# Autodesk Inventor assembly: leg_right
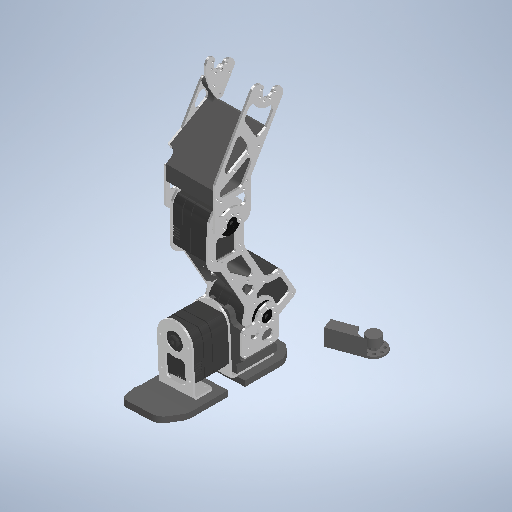
[picture p0: Inventor's stored thumbnail of the model, 512x512]
Saved by Autodesk Inventor 2026.1 (Build 301233020, 233B)
## iProperties
Created: 2024-10-11
Part Number: leg_right
Document SubType Name: Assembly
Designer: hibik
Author: hibik
## Documents named in this file (5)
- C:\Users\hibik\Documents\Robomech\HR\Eglantyne_mark2\hard\leg\leg_right.iam
- C:\Users\hibik\Documents\Robomech\HR\Eglantyne_mark2\hard\leg\leg_upper_right.iam
- C:\Users\hibik\Documents\Robomech\HR\Eglantyne_mark2\hard\leg\leg_under.iam
- C:\Users\hibik\Documents\Robomech\HR\Eglantyne_mark2\hard\leg\toe.iam
- C:\Users\hibik\Documents\Robomech\HR\Eglantyne_mark2\hard\leg\spring_setter\axis.ipt
## Components (4 placed, 4 different names)
1. leg_upper_right:1 [sub-assembly] — 挿入:1
2. leg_under:1 [sub-assembly] — 挿入:1, 挿入:2
3. toe:1 [sub-assembly] — 挿入:2
4. axis:1
## Relationships (2: Insert 2)
- 挿入:1 [Insert]: leg_upper_right:1 ↔ leg_under:1
- 挿入:2 [Insert]: leg_under:1 ↔ toe:1
